# Autodesk Inventor assembly: node
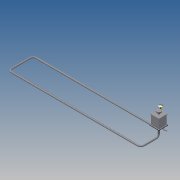
[picture p0: Inventor's stored thumbnail of the model, 180x180]
Saved by Autodesk Inventor 2014 SP1 (Build 180222100, 222)
## iProperties
Created: 2014-03-11
Part Number: node
Document SubType Name: Assembly
Designer: Dave
Author: Dave
## Documents named in this file (16)
- C:\Users\Dave\Desktop\hera-cad\Node\node.iam
- C:\Users\Dave\Desktop\hera-cad\Node\plinth.ipt
- C:\Users\Dave\Desktop\hera-cad\Node\housing.ipt
- C:\Users\Dave\Desktop\hera-cad\Node\snap.ipt
- C:\Users\Dave\Desktop\hera-cad\Node\Acopian-M13-Case.iam
- C:\Users\Dave\Desktop\hera-cad\Node\undergroundPipe.iam
- C:\Users\Dave\Desktop\hera-cad\Node\Ground.ipt
- C:\Users\Dave\Desktop\hera-cad\Node\frameAssembly.iam
- C:\Users\Dave\Desktop\hera-cad\Node\pam.ipt
- C:\Users\Dave\Desktop\hera-cad\Node\housingLidAssembly.iam
- C:\Users\Dave\Desktop\hera-cad\Node\innerHousingAssembly.iam
- C:\Users\Dave\Desktop\hera-cad\Node\chimney.ipt
- C:\Users\Dave\Desktop\PAPER\2013deploy\containerBulkheadAssy.iam
- C:\Users\Dave\Desktop\hera-cad\Node\inlineFan.ipt
- C:\Users\Dave\Desktop\hera-cad\Node\sweep_4in.ipt
- C:\Users\Dave\Desktop\hera-cad\Node\node\AIP\Cable and Harness\node.Power.iam
## Components (38 placed, 15 different names)
1. plinth:1 — Mate:1, Mate:7, toPlinth, Insert:10, Insert:11
2. housing:1 — Mate:1, Mate:13, Mate:21, Flush:8, Mate:24, Mate:25
3. Ground:1 — Mate:7
4. frameAssembly:1 [sub-assembly] — Mate:14, Flush:5, Mate:15, Mate:16, Flush:6, Mate:17, Mate:18, Flush:7, Mate:19, toPlinth, Mate:23
5. housingLidAssembly:1 [sub-assembly] — Mate:25
6. innerHousingAssembly:1 [sub-assembly] — Mate:23
7. containerBulkheadAssy:1 [sub-assembly] — Mate:24
8. undergroundPipe:1 [sub-assembly] — Insert:11, Insert:12
9. inlineFan:1 — Insert:9, Insert:12
10. chimney:1 — Insert:9
11. sweep_4in:1 — Insert:10
12. node.Power [sub-assembly]
13. pam:1 — Mate:16, Flush:6, Mate:17
14. pam:2
15. pam:3
16. pam:4
17. pam:5
18. pam:6
19. pam:7
20. pam:8
21. pam:9
22. pam:10 — Mate:14, Flush:5, Mate:15
23. pam:11
24. pam:12
25. pam:13
26. pam:14
27. pam:15
28. pam:16
29. pam:17
30. pam:18
31. snap:1 — Mate:18, Flush:7, Mate:19
32. snap:2
33. snap:3
34. snap:4
35. snap:5
36. snap:6
37. Acopian-M13-Case:1 [sub-assembly] — Mate:13, Mate:21, Flush:8
38. Acopian-M13-Case:2 [sub-assembly]
## Component patterns: pam2 (9 elements), pam1 (9 elements), snap (6 elements), analogPower (2 elements)
## Relationships (22: Mate 14, Flush 4, Insert 4)
- Mate:1: plinth:1 ↔ housing:1
- Mate:7: plinth:1 ↔ Ground:1
- Mate:13 (5.08 mm): housing:1 ↔ Acopian-M13-Case:1
- Mate:14: frameAssembly:1 ↔ pam:10
- Flush:5: frameAssembly:1 ↔ pam:10
- Mate:15 (50.8 mm): frameAssembly:1 ↔ pam:10
- Mate:16: frameAssembly:1 ↔ pam:1
- Flush:6: frameAssembly:1 ↔ pam:1
- Mate:17 (50.8 mm): frameAssembly:1 ↔ pam:1
- Mate:18: frameAssembly:1 ↔ snap:1
- Flush:7: frameAssembly:1 ↔ snap:1
- Mate:19 (76.2 mm): frameAssembly:1 ↔ snap:1
- toPlinth [Mate]: plinth:1 ↔ frameAssembly:1
- Mate:21 (203.2 mm): housing:1 ↔ Acopian-M13-Case:1
- Flush:8 (406.4 mm): housing:1 ↔ Acopian-M13-Case:1
- Mate:23: frameAssembly:1 ↔ innerHousingAssembly:1
- Mate:24: housing:1 ↔ containerBulkheadAssy:1
- Insert:9: inlineFan:1 ↔ chimney:1
- Insert:10: plinth:1 ↔ sweep_4in:1
- Insert:11: plinth:1 ↔ undergroundPipe:1
- Insert:12: undergroundPipe:1 ↔ inlineFan:1
- Mate:25: housing:1 ↔ housingLidAssembly:1
